# Autodesk Inventor assembly: BALL SCREW ASSEMBLY
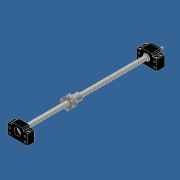
[picture p0: Inventor's stored thumbnail of the model, 180x180]
Saved by Autodesk Inventor 2013 SP2 (Build 170200200, 200)
## iProperties
Created: 2013-04-30
Part Number: BALL SCREW ASSEMBLY
Document SubType Name: Assembly
Designer: J.WASSERSTRASS
Mass: 677.375 g
Surface Area: 645.281 cm^2
Volume: 134.942 cm^3
Density: 5.01975 g/cm^3
TRAVEL_LIMIT: 0.100 in
Author: J.WASSERSTRASS
## Documents named in this file (7)
- \\kitt\Users\jeremy_wasserstrass\Personal projects\cnc-printer\mechanical\design\BALL SCREW ASSEMBLY.iam
- \\kitt\Users\jeremy_wasserstrass\Personal projects\cnc-printer\mechanical\design\1204 BALL NUT.ipt
- \\kitt\Users\jeremy_wasserstrass\Personal projects\cnc-printer\mechanical\design\1204 BALL SCREW.ipt
- \\kitt\Users\jeremy_wasserstrass\Personal projects\cnc-printer\mechanical\design\BF10 BEARING BLOCK.ipt
- \\kitt\Users\jeremy_wasserstrass\Personal projects\cnc-printer\mechanical\design\BK10 BEARING BLOCK.ipt
- \\kitt\Users\jeremy_wasserstrass\Personal projects\cnc-printer\mechanical\design\Imported Components\5972K286\5972K286.ipt
- \\kitt\Users\jeremy_wasserstrass\Personal projects\cnc-printer\mechanical\design\MMC 6661K820 8mm ID BEARING.ipt
## Components (7 placed, 6 different names)
1. 1204 BALL NUT:1 — Mate:1, TRAVEL LIMITS
2. 1204 BALL SCREW:1 — Mate:1, Insert:6, Insert:10
3. BF10 BEARING BLOCK:1 — Flush:1, TRAVEL LIMITS, Insert:9
4. BK10 BEARING BLOCK:1 — Flush:1, Insert:6, Insert:7, Insert:8
5. 5972K286:2 — Insert:7
6. 5972K286:3 — Insert:8
7. MMC 6661K820 8mm ID BEARING:1 — Insert:9, Insert:10
## Relationships (8: Insert 5, Mate 2, Flush 1)
- Mate:1: 1204 BALL NUT:1 ↔ 1204 BALL SCREW:1
- Flush:1: BF10 BEARING BLOCK:1 ↔ BK10 BEARING BLOCK:1
- TRAVEL LIMITS [Mate] (2.54 mm): 1204 BALL NUT:1 ↔ BF10 BEARING BLOCK:1
- Insert:6: 1204 BALL SCREW:1 ↔ BK10 BEARING BLOCK:1
- Insert:7: BK10 BEARING BLOCK:1 ↔ 5972K286:2
- Insert:8 (1 mm): BK10 BEARING BLOCK:1 ↔ 5972K286:3
- Insert:9: BF10 BEARING BLOCK:1 ↔ MMC 6661K820 8mm ID BEARING:1
- Insert:10: 1204 BALL SCREW:1 ↔ MMC 6661K820 8mm ID BEARING:1
## Named parameters: TRAVEL_LIMIT = 2.54 mm
